# Autodesk Inventor assembly: complete setup met relief
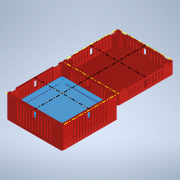
[picture p0: Inventor's stored thumbnail of the model, 180x180]
Saved by Autodesk Inventor 2021 (Build 250183000, 183)
## iProperties
Created: 2023-11-13
Part Number: complete setup met relief
Document SubType Name: Assembly
Designer: Elias
Author: Elias
## Documents named in this file (5)
- D:\Hoge school ICT\2.0 Project experience 2.1\Tekeningen\13_11_2023\complete setup met relief.iam
- D:\Hoge school ICT\2.0 Project experience 2.1\Tekeningen\13_11_2023\Led behuizing dubbele hoogte.ipt
- D:\Hoge school ICT\2.0 Project experience 2.1\Tekeningen\13_11_2023\Led deksel niet hub.ipt
- D:\Hoge school ICT\2.0 Project experience 2.1\Tekeningen\13_11_2023\ledstrip.ipt
- D:\Hoge school ICT\2.0 Project experience 2.1\Tekeningen\13_11_2023\Led behuizing.ipt
## Components (7 placed, 4 different names)
1. Led behuizing dubbele hoogte:1 — Mate:1, Mate:2, Mate:10, Flush:7, Flush:8, Mate:11
2. Led deksel niet hub:1 — Mate:1, Mate:2, Mate:3, Mate:4, Mate:5, Mate:6, Flush:2, Flush:3, Flush:4, Flush:5, Flush:6, Mate:11
3. ledstrip:1 — Mate:6, Flush:3, Flush:6, Mate:7
4. ledstrip:2 — Mate:5, Flush:2, Mate:7, Mate:8
5. ledstrip:3 — Mate:3, Flush:5, Mate:9
6. ledstrip:4 — Mate:4, Flush:4, Mate:8, Mate:9
7. Led behuizing:1 — Mate:10, Flush:7, Flush:8
## Relationships (18: Mate 11, Flush 7)
- Mate:1: Led behuizing dubbele hoogte:1 ↔ Led deksel niet hub:1
- Mate:2: Led behuizing dubbele hoogte:1 ↔ Led deksel niet hub:1
- Mate:3: Led deksel niet hub:1 ↔ ledstrip:3
- Mate:4: Led deksel niet hub:1 ↔ ledstrip:4
- Mate:5: Led deksel niet hub:1 ↔ ledstrip:2
- Mate:6: Led deksel niet hub:1 ↔ ledstrip:1
- Flush:2 (32 mm): Led deksel niet hub:1 ↔ ledstrip:2
- Flush:3 (32 mm): Led deksel niet hub:1 ↔ ledstrip:1
- Flush:4 (32 mm): Led deksel niet hub:1 ↔ ledstrip:4
- Flush:5 (32 mm): Led deksel niet hub:1 ↔ ledstrip:3
- Flush:6 (25 mm): Led deksel niet hub:1 ↔ ledstrip:1
- Mate:7 (20 mm): ledstrip:1 ↔ ledstrip:2
- Mate:8 (20 mm): ledstrip:2 ↔ ledstrip:4
- Mate:9 (20 mm): ledstrip:3 ↔ ledstrip:4
- Mate:10: Led behuizing dubbele hoogte:1 ↔ Led behuizing:1
- Flush:7: Led behuizing dubbele hoogte:1 ↔ Led behuizing:1
- Flush:8: Led behuizing dubbele hoogte:1 ↔ Led behuizing:1
- Mate:11: Led behuizing dubbele hoogte:1 ↔ Led deksel niet hub:1
